# Autodesk Inventor assembly: Robot_Base
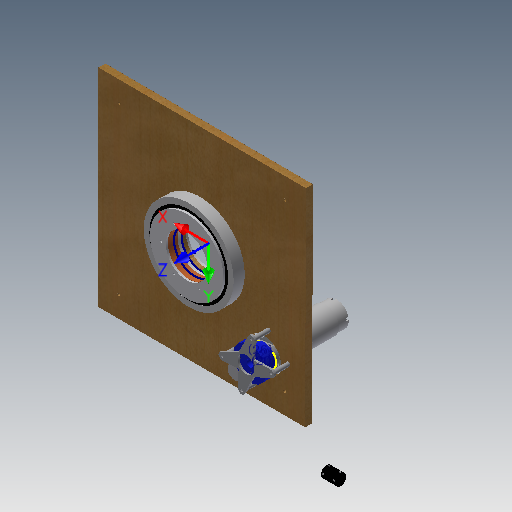
[picture p0: Inventor's stored thumbnail of the model, 512x512]
Saved by Autodesk Inventor 2019.4 (Build 234330000, 330)
## iProperties
Created: 2018-08-09
Part Number: Robot_Base
Document SubType Name: Assembly
Designer: Owner
Mass: 868.193 g
Surface Area: 3500.78 cm^2
Volume: 1203.12 cm^3
Density: 0.72162 g/cm^3
Author: Owner
## Documents named in this file (18)
- E:\ロボ研\キャチロボ\キャチロボ2019\加工指示用\2019-6-17_HDarm\Robot_Base.iam
- E:\ロボ研\キャチロボ\キャチロボ2019\加工指示用\2019-6-17_HDarm\ベアリングRB9016UUCOO.ipt
- E:\ロボ研\キャチロボ\キャチロボ2019\加工指示用\2019-6-17_HDarm\ベアリン押さえ.ipt
- E:\ロボ研\キャチロボ\キャチロボ2019\加工指示用\2019-6-17_HDarm\アーム支え板1.ipt
- E:\ロボ研\キャチロボ\キャチロボ2019\加工指示用\2019-6-17_HDarm\アームベース下円盤.ipt
- E:\ロボ研\キャチロボ\キャチロボ2019\加工指示用\2019-6-17_HDarm\RS555PH_Geared_Motor.ipt
- E:\ロボ研\キャチロボ\キャチロボ2019\加工指示用\2019-6-17_HDarm\PS1-48.ipt
- E:\ロボ研\キャチロボ\キャチロボ2019\加工指示用\2019-6-17_HDarm\ベアリング押さえアルミ.ipt
- E:\ロボ研\キャチロボ\キャチロボ2019\加工指示用\2019-6-17_HDarm\RS555マウント.ipt
- E:\ロボ研\キャチロボ\キャチロボ2019\加工指示用\2019-6-17_HDarm\D留め板.ipt
- E:\ロボ研\キャチロボ\キャチロボ2019\加工指示用\2019-6-17_HDarm\ギア支え1.ipt
- E:\ロボ研\キャチロボ\キャチロボ2019\加工指示用\2019-6-17_HDarm\φ6スペーサ1.ipt
- E:\ロボ研\キャチロボ\キャチロボ2019\加工指示用\2019-6-17_HDarm\MCJN16-6-6.iam
- E:\ロボ研\キャチロボ\キャチロボ2019\加工指示用\2019-6-17_HDarm\E6A2_CWZ3C.ipt
- E:\ロボ研\キャチロボ\キャチロボ2019\加工指示用\2019-6-17_HDarm\MCJN14-4-4.iam
- E:\ロボ研\キャチロボ\キャチロボ2019\加工指示用\2019-6-17_HDarm\DfixPit.ipt
- E:\ロボ研\キャチロボ\キャチロボ2019\加工指示用\2019-6-17_HDarm\2axsisSensGear.ipt
- E:\ロボ研\キャチロボ\キャチロボ2019\加工指示用\2019-6-17_HDarm\ロボットベース2019.ipt
## Components (20 placed, 17 different names)
1. ベアリングRB9016UUCOO:1 — 回転:7
2. ロボットベース2018:1 — 回転:2, 回転:3, 回転:4, 回転:5, メイト:11, メイト:12, 挿入:2, 回転:6, リジッド:3
3. アーム支え板1:1 — 回転:6
4. アームベース下円盤:1 — リジッド:3, 回転:7, 回転:8
5. RS555PH_Geared_Motor:1 — メイト:4, リジッド:1, リジッド:2, メイト:9, 挿入:2
6. PS1-48:1 — メイト:4, メイト:7, メイト:8, メイト:10, メイト:12
7. ベアリング押さえアルミ:1 — 回転:9
8. RS555マウント:1 — メイト:9
9. D留め板:1 — リジッド:1, メイト:8
10. ギア支え1:1 — メイト:1
11. φ6スペーサ1:1 — メイト:1, 回転:2
12. MCJN16-6-6:1 [sub-assembly]
13. E6A2_CWZ3C:1 — 回転:1
14. MCJN14-4-4:1 [sub-assembly] — 回転:1, 挿入:1
15. DfixPit:1 — リジッド:2, メイト:7
16. 2axsisSensGear:1 — 挿入:1, メイト:10, メイト:11
17. φ6スペーサ1:2 — 回転:5
18. φ6スペーサ1:3 — 回転:4
19. φ6スペーサ1:4 — 回転:3
20. ベアリン押さえ:2 — 回転:8, 回転:9
## Relationships (22: RevoluteJoint 9, Mate 8, WeldJoint 3, Insert 2)
- 回転:1 [RevoluteJoint]: E6A2_CWZ3C:1 ↔ MCJN14-4-4:1
- メイト:1 [Mate]: ギア支え1:1 ↔ φ6スペーサ1:1
- メイト:4 [Mate]: RS555PH_Geared_Motor:1 ↔ PS1-48:1
- リジッド:1 [WeldJoint]: RS555PH_Geared_Motor:1 ↔ D留め板:1
- リジッド:2 [WeldJoint]: RS555PH_Geared_Motor:1 ↔ DfixPit:1
- メイト:7 [Mate]: PS1-48:1 ↔ DfixPit:1
- メイト:8 [Mate]: PS1-48:1 ↔ D留め板:1
- メイト:9 [Mate]: RS555PH_Geared_Motor:1 ↔ RS555マウント:1
- 挿入:1 [Insert] (30 mm): MCJN14-4-4:1 ↔ 2axsisSensGear:1
- メイト:10 [Mate] (34 mm): PS1-48:1 ↔ 2axsisSensGear:1
- 回転:2 [RevoluteJoint]: ロボットベース2018:1 ↔ φ6スペーサ1:1
- 回転:3 [RevoluteJoint]: ロボットベース2018:1 ↔ φ6スペーサ1:4
- 回転:4 [RevoluteJoint]: ロボットベース2018:1 ↔ φ6スペーサ1:3
- 回転:5 [RevoluteJoint]: ロボットベース2018:1 ↔ φ6スペーサ1:2
- メイト:11 [Mate]: ロボットベース2018:1 ↔ 2axsisSensGear:1
- メイト:12 [Mate]: ロボットベース2018:1 ↔ PS1-48:1
- 挿入:2 [Insert] (3 mm): ロボットベース2018:1 ↔ RS555PH_Geared_Motor:1
- 回転:6 [RevoluteJoint]: ロボットベース2018:1 ↔ アーム支え板1:1
- リジッド:3 [WeldJoint]: ロボットベース2018:1 ↔ アームベース下円盤:1
- 回転:7 [RevoluteJoint]: ベアリングRB9016UUCOO:1 ↔ アームベース下円盤:1
- 回転:8 [RevoluteJoint]: アームベース下円盤:1 ↔ ベアリン押さえ:2
- 回転:9 [RevoluteJoint]: ベアリング押さえアルミ:1 ↔ ベアリン押さえ:2
